# Autodesk Inventor assembly: dome with double door
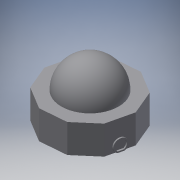
[picture p0: Inventor's stored thumbnail of the model, 180x180]
Saved by Autodesk Inventor 2017 (Build 210142000, 142)
## iProperties
Created: 2018-03-14
Part Number: dome with double door
Document SubType Name: Assembly
Designer: braxtonwright
Author: braxtonwright
## Documents named in this file (3)
- D:\School\Game develpment\geoscape\rooms\assembly\dome with double door.iam
- D:\School\Game develpment\geoscape\rooms\dome.ipt
- D:\School\Game develpment\geoscape\doors\double door.ipt
## Components (2 placed, 2 different names)
1. dome:1 — Mate:1, Mate:2, Mate:3
2. double door:1 — Mate:1, Mate:2, Mate:3
## Relationships (3: Mate 3)
- Mate:1: dome:1 ↔ double door:1
- Mate:2: dome:1 ↔ double door:1
- Mate:3: dome:1 ↔ double door:1
